# Autodesk Inventor assembly: ShooterWheelSub
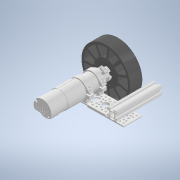
[picture p0: Inventor's stored thumbnail of the model, 180x180]
Saved by Autodesk Inventor 2020 (Build 240168000, 168)
## iProperties
Created: 2021-02-27
Part Number: ShooterWheelSub
Document SubType Name: Assembly
Designer: tdmp4
Author: tdmp4
## Documents named in this file (8)
- C:\Users\tdmp4\OneDrive\Documents\GitHub\CAD-2021-Ultimate_Goal\Shooter\ShooterWheelSub.iam
- C:\Users\tdmp4\OneDrive\Documents\GitHub\CAD-2021-Ultimate_Goal\ServoCity\565022.ipt
- C:\Users\tdmp4\OneDrive\Documents\GitHub\CAD-2021-Ultimate_Goal\ServoCity\585720.ipt
- C:\Users\tdmp4\OneDrive\Documents\GitHub\CAD-2021-Ultimate_Goal\ServoCity\555176 assembly.ipt
- C:\Users\tdmp4\OneDrive\Documents\GitHub\CAD-2021-Ultimate_Goal\GoBilda\5202-0002-0014 part.ipt
- C:\Users\tdmp4\OneDrive\Documents\GitHub\CAD-2021-Ultimate_Goal\ServoCity\545618 assembly.ipt
- C:\Users\tdmp4\OneDrive\Documents\GitHub\CAD-2021-Ultimate_Goal\AndyMark\am-3563 4IN 8mm Round Compliant Wheel REV2.ipt
- C:\Users\tdmp4\OneDrive\Documents\GitHub\CAD-2021-Ultimate_Goal\ServoCity\545456.ipt
## Components (9 placed, 7 different names)
1. 565022:1 — Mate:3, Flush:7, Flush:8
2. 585720:1 — Mate:3, Flush:7, Flush:8, Mate:4, Mate:5, Mate:6
3. 585720:2 — Mate:4, Mate:5, Mate:6, Mate:7, Mate:8, Mate:9, Mate:10, Mate:11, Mate:12
4. 555176 assembly:1 — Mate:10, Mate:11, Mate:12
5. 555176 assembly:2 — Mate:7, Mate:8, Mate:9, Mate:13, Mate:14
6. 5202-0002-0014 part:1 — Mate:13, Mate:14, Mate:20, Mate:21
7. 545618 assembly:1 — Mate:17, Mate:18, Mate:19, Mate:20, Mate:21
8. am-3563 4IN 8mm Round Compliant Wheel REV2:1 — Mate:15, Mate:16
9. 545456:1 — Mate:15, Mate:16, Mate:17, Mate:18, Mate:19
## Relationships (21: Mate 19, Flush 2)
- Mate:3: 565022:1 ↔ 585720:1
- Flush:7: 565022:1 ↔ 585720:1
- Flush:8 (14.9606 mm): 565022:1 ↔ 585720:1
- Mate:4: 585720:1 ↔ 585720:2
- Mate:5: 585720:1 ↔ 585720:2
- Mate:6: 585720:1 ↔ 585720:2
- Mate:7: 585720:2 ↔ 555176 assembly:2
- Mate:8: 585720:2 ↔ 555176 assembly:2
- Mate:9: 585720:2 ↔ 555176 assembly:2
- Mate:10: 585720:2 ↔ 555176 assembly:1
- Mate:11: 585720:2 ↔ 555176 assembly:1
- Mate:12: 585720:2 ↔ 555176 assembly:1
- Mate:13: 555176 assembly:2 ↔ 5202-0002-0014 part:1
- Mate:14: 555176 assembly:2 ↔ 5202-0002-0014 part:1
- Mate:15: am-3563 4IN 8mm Round Compliant Wheel REV2:1 ↔ 545456:1
- Mate:16: am-3563 4IN 8mm Round Compliant Wheel REV2:1 ↔ 545456:1
- Mate:17: 545618 assembly:1 ↔ 545456:1
- Mate:18: 545618 assembly:1 ↔ 545456:1
- Mate:19: 545618 assembly:1 ↔ 545456:1
- Mate:20: 5202-0002-0014 part:1 ↔ 545618 assembly:1
- Mate:21: 5202-0002-0014 part:1 ↔ 545618 assembly:1
